# Autodesk Inventor assembly: Wheel
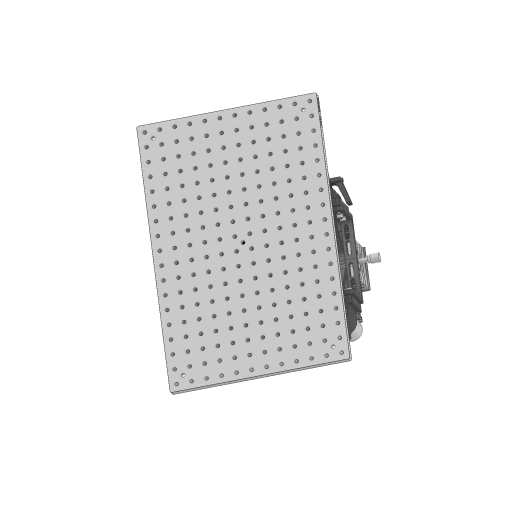
[picture p0: Inventor's stored thumbnail of the model, 512x512]
Saved by Autodesk Inventor 2024.1 (Build 281209000, 209)
## iProperties
Created: 2021-11-12
Part Number: Wheel
Document SubType Name: Assembly
Designer: gnzak
Author: gnzak
Comments: Wheel (spokes, track, clamp, axle, bearings): 0.306 lb Top Gonio: 0.661 Pillar: 3.73 Adjustable clamp: 1.09 3 5" t-slot rails: 0.624 brackets: 0.273 head bars: 1.02 wheel: 0.306 Total: 7.704 lb Max Capacity of bottom gonio: 6.61 16% over capacity
## Documents named in this file (29)
- C:\Users\rosam\Documents\repos\vr-frame-l7.033\Assemblies\Wheel_on-board_rotatable_original-headbars_adjustable.iam
- C:\Users\rosam\Documents\repos\vr-frame-l7.033\Parts\ThorLabs RA180\RA180.ipt
- C:\Users\rosam\Documents\repos\vr-frame-l7.033\Parts\ThorLabs PH1\PH1.ipt
- C:\Users\rosam\Documents\repos\vr-frame-l7.033\Parts\ThorLabs MB1218\MB1218 - Aluminium Breadboard 304.8 x 457.2 x 12.7mm_MB3030_M-1.ipt
- C:\Users\rosam\Documents\repos\vr-frame-l7.033\Parts\McMaster-Carr 47065T595\47065T595_Red Plastic Pull Handle.ipt
- C:\Users\rosam\Documents\repos\vr-frame-l7.033\Parts\ThorLabs TR6\TR6-Step.ipt
- C:\Users\rosam\Documents\repos\vr-frame-l7.033\Parts\ThorLabs TR12\TR12-Step.ipt
- C:\Users\rosam\Documents\repos\vr-frame-l7.033\Parts\ThorLabs TR2\TR2.ipt
- C:\Users\rosam\Documents\repos\vr-frame-l7.033\Parts\ThorLabs TR3\TR3-Step.ipt
- C:\Users\rosam\Documents\repos\vr-frame-l7.033\Parts\ThorLabs RA90\RA90-Step.ipt
- C:\Users\rosam\Documents\repos\vr-frame-l7.033\Parts\ThorLabs VH1\VH1-Step.ipt
- C:\Users\rosam\Documents\repos\vr-frame-l7.033\Parts\Parker Series 3 - Miniature Inert Liquid Valve\Series 3 (2way, .062Barb)-shell.ipt
- C:\Users\rosam\Documents\repos\vr-frame-l7.033\Parts\Solenoid Holder\Solenoid Mounting Panel.ipt
- C:\Users\rosam\Documents\repos\vr-frame-l7.033\Parts\McMaster-Carr 47065T801\47065T801_T-Slotted Framing_5-inches.ipt
- C:\Users\rosam\Documents\repos\vr-frame-l7.033\Parts\McMaster-Carr 47065T236\47065T236_Silver Corner Bracket.ipt
- C:\Users\rosam\Documents\repos\vr-frame-l7.033\Assemblies\Goniometers_70x70.iam
- C:\Users\rosam\Documents\repos\vr-frame-l7.033\Parts\Thorlabs C1515\C1515.ipt
- C:\Users\rosam\Documents\repos\vr-frame-l7.033\Parts\ThorLabs DP8A\DP8A-Step.ipt
- C:\Users\rosam\Documents\repos\vr-frame-l7.033\Parts\McMaster-Carr 47065T239\47065T239_Silver Corner Bracket.ipt
- C:\Users\rosam\Documents\repos\vr-frame-l7.033\Parts\McMaster-Carr 3136N157\3136N157_T-Slotted Framing.ipt
- C:\Users\rosam\Documents\repos\vr-frame-l7.033\Parts\McMaster-Carr 3136N175\3136N175_T-Slotted Framing.ipt
- C:\Users\rosam\Documents\repos\vr-frame-l7.033\Assemblies\Wheel.iam
- C:\Users\rosam\Documents\repos\vr-frame-l7.033\Parts\McMaster-Carr 47065T801\47065T801_T-Slotted Framing_4.4-inches.ipt
- C:\Users\rosam\Documents\repos\vr-frame-l7.033\Parts\McMaster-Carr 47065T255\47065T255_T-Slotted Framing.ipt
- C:\Users\rosam\Documents\repos\vr-frame-l7.033\Assemblies\bearing holder w bearing (vr).iam
- C:\Users\rosam\Documents\repos\vr-frame-l7.033\Assemblies\VR Head Bar Holder Left.iam
- C:\Users\rosam\Documents\repos\vr-frame-l7.033\Assemblies\VR Head Bar Holder Right.iam
- C:\Users\rosam\Documents\repos\vr-frame-l7.033\Parts\McMaster_Shaft-Coupler_6412K11\Shaft-Coupler_6412K11.ipt
- C:\Users\rosam\Documents\repos\vr-frame-l7.033\Parts\McMaster_Rotary-Shaft\6061K101_Linear Motion Shaft.ipt
## Components (44 placed, 28 different names)
1. MB1218 - Aluminium Breadboard 304.8 x 457.2 x 12.7mm_MB3030_M-1:1 — Angle:1, Mate:54, Mate:55, Mate:56, Mate:58, Mate:59, Mate:83, Mate:85, Mate:89, Angle:4, Angle:7, Mate:98, Angle:12, Angle:27, Mate:155, Mate:193, Mate:194, Angle:34, Angle:35, Mate:254, Mate:255, Mate:256, Angle:38, Angle:41, Mate:274, Mate:309, Angle:49, Mate:310, Angle:50
2. 47065T595_Red Plastic Pull Handle:1 — Mate:54, Mate:56, Mate:57, Mate:59
3. 47065T595_Red Plastic Pull Handle:2 — Mate:55, Mate:57, Mate:58
4. PH1:3 — Mate:85, Mate:89, Angle:7, Mate:97
5. PH1:5 — Mate:83, Angle:4, Mate:153, Mate:154
6. TR6-Step:4 — Mate:106, Mate:107, Mate:153, Mate:154, Mate:155
7. TR12-Step:1 — Mate:95, Mate:96, Mate:97, Mate:98
8. TR2:1 — Mate:95, Mate:96, Mate:99, Mate:100
9. RA180:3 — Mate:99, Mate:100, Mate:101, Mate:102, Angle:9, Angle:10
10. TR3-Step:1 — Mate:101, Mate:102, Mate:103, Flush:9, Mate:104, Flush:10
11. RA90-Step:1 — Mate:104, Flush:10, Angle:10
12. RA90-Step:2 — Mate:103, Flush:9, Angle:9, Angle:27
13. VH1-Step:1 — Mate:106, Angle:12, Mate:107
14. Series 3 (2way, .062Barb)-shell:3 — Mate:134, Angle:25, Mate:136, Mate:199
15. Series 3 (2way, .062Barb)-shell:4 — Mate:133, Mate:135, Angle:24, Mate:200
16. Solenoid Mounting Panel:2 — Mate:133, Mate:134, Mate:135, Angle:24, Angle:25, Mate:136, Mate:195, Mate:196, Angle:35
17. 47065T801_T-Slotted Framing_5-inches:1 — Mate:193, Mate:194, Angle:34, Mate:195, Mate:196, Mate:197, Mate:198, Flush:29, Flush:30
18. 47065T236_Silver Corner Bracket:1 — Mate:197, Mate:200, Flush:30
19. 47065T236_Silver Corner Bracket:2 — Mate:198, Mate:199, Flush:29
20. Goniometers_70x70:1 [sub-assembly] — Angle:38, Mate:262, Mate:276, Mate:277, Mate:280, Mate:281, Mate:282, Mate:303, Mate:305, Flush:78
21. 47065T801_T-Slotted Framing_5-inches:2 — Mate:248, Mate:252, Flush:47, Mate:298, Flush:57, Flush:58, Flush:62, Mate:302, Flush:63, Flush:64, Mate:316, Flush:71, Flush:72, Mate:321, Mate:325
22. 47065T801_T-Slotted Framing_5-inches:3 — Mate:250, Mate:253, Flush:49, Mate:299, Flush:59, Flush:60, Flush:61, Mate:314, Flush:67, Flush:68, Mate:315, Flush:69, Flush:70, Mate:323, Flush:79
23. C1515:2 — Mate:241, Flush:51, Mate:275, Flush:52, Mate:280, Flush:76
24. DP8A-Step:1 — Mate:241, Mate:254, Mate:255, Mate:256, Flush:76
25. 47065T239_Silver Corner Bracket:1 — Mate:248, Mate:298, Flush:57, Flush:58
26. 47065T239_Silver Corner Bracket:2 — Mate:250, Mate:299, Flush:59, Flush:60
27. 3136N157_T-Slotted Framing:1 — Mate:252, Flush:47, Flush:62, Mate:322
28. 3136N157_T-Slotted Framing:2 — Mate:253, Flush:49, Flush:61, Mate:324
29. 3136N175_T-Slotted Framing:1 — Mate:262, Mate:276, Mate:277, Mate:304
30. Wheel:1 [sub-assembly] — Tangent:1, Tangent:2, Flush:78
31. C1515:3 — Angle:41, Flush:51, Mate:275, Flush:52, Mate:281, Mate:282
32. DP8A-Step:2 — Mate:274
33. 47065T801_T-Slotted Framing_4.4-inches:1 — Mate:302, Flush:63, Flush:64, Mate:303, Mate:304, Mate:305, Mate:314, Flush:67, Flush:68
34. VH1-Step:2 — Mate:312, Mate:313
35. 47065T255_T-Slotted Framing:1 — Mate:309, Angle:49, Mate:310, Mate:311, Flush:65, Flush:66
36. 47065T801_T-Slotted Framing_5-inches:6 — Mate:311, Flush:65, Flush:66, Mate:312, Mate:313
37. 47065T801_T-Slotted Framing_5-inches:7 — Mate:316, Flush:71, Flush:72, Mate:317, Flush:73
38. 47065T801_T-Slotted Framing_5-inches:8 — Mate:315, Flush:69, Flush:70, Mate:318, Flush:74
39. bearing holder w bearing (vr):1 [sub-assembly] — Mate:317, Flush:73, Flush:75, Mate:327, Flush:80
40. bearing holder w bearing (vr):2 [sub-assembly] — Mate:318, Flush:74, Flush:75, Mate:326
41. VR Head Bar Holder Left:1 [sub-assembly] — Mate:321, Mate:322, Mate:325
42. VR Head Bar Holder Right:1 [sub-assembly] — Mate:323, Mate:324, Flush:79, Mate:326
43. Shaft-Coupler_6412K11:1 — Mate:328, Angle:50, Flush:81
44. 6061K101_Linear Motion Shaft:1 — Mate:327, Flush:80, Mate:328, Flush:81
## Relationships (131: Mate 79, Flush 33, Angle 17, Tangent 2)
- Angle:1 (0 deg): MB1218 - Aluminium Breadboard 304.8 x 457.2 x 12.7mm_MB3030_M-1:1
- Flush:6 (25.4 mm)
- Mate:54: MB1218 - Aluminium Breadboard 304.8 x 457.2 x 12.7mm_MB3030_M-1:1 ↔ 47065T595_Red Plastic Pull Handle:1
- Mate:55: MB1218 - Aluminium Breadboard 304.8 x 457.2 x 12.7mm_MB3030_M-1:1 ↔ 47065T595_Red Plastic Pull Handle:2
- Mate:56: MB1218 - Aluminium Breadboard 304.8 x 457.2 x 12.7mm_MB3030_M-1:1 ↔ 47065T595_Red Plastic Pull Handle:1
- Mate:57: 47065T595_Red Plastic Pull Handle:1 ↔ 47065T595_Red Plastic Pull Handle:2
- Mate:58 (-12.7 mm): MB1218 - Aluminium Breadboard 304.8 x 457.2 x 12.7mm_MB3030_M-1:1 ↔ 47065T595_Red Plastic Pull Handle:2
- Mate:59 (-12.7 mm): MB1218 - Aluminium Breadboard 304.8 x 457.2 x 12.7mm_MB3030_M-1:1 ↔ 47065T595_Red Plastic Pull Handle:1
- Mate:83: MB1218 - Aluminium Breadboard 304.8 x 457.2 x 12.7mm_MB3030_M-1:1 ↔ PH1:5
- Mate:85: MB1218 - Aluminium Breadboard 304.8 x 457.2 x 12.7mm_MB3030_M-1:1 ↔ PH1:3
- Mate:89: MB1218 - Aluminium Breadboard 304.8 x 457.2 x 12.7mm_MB3030_M-1:1 ↔ PH1:3
- Angle:4 (0 deg): MB1218 - Aluminium Breadboard 304.8 x 457.2 x 12.7mm_MB3030_M-1:1 ↔ PH1:5
- Angle:7 (0 deg): MB1218 - Aluminium Breadboard 304.8 x 457.2 x 12.7mm_MB3030_M-1:1 ↔ PH1:3
- Mate:95: TR12-Step:1 ↔ TR2:1
- Mate:96: TR12-Step:1 ↔ TR2:1
- Mate:97: PH1:3 ↔ TR12-Step:1
- Mate:98: MB1218 - Aluminium Breadboard 304.8 x 457.2 x 12.7mm_MB3030_M-1:1 ↔ TR12-Step:1
- Mate:99: TR2:1 ↔ RA180:3
- Mate:100: TR2:1 ↔ RA180:3
- Mate:101: RA180:3 ↔ TR3-Step:1
- Mate:102: RA180:3 ↔ TR3-Step:1
- Mate:103: TR3-Step:1 ↔ RA90-Step:2
- Flush:9: TR3-Step:1 ↔ RA90-Step:2
- Angle:9 (0 deg): RA180:3 ↔ RA90-Step:2
- Mate:104: TR3-Step:1 ↔ RA90-Step:1
- Flush:10: TR3-Step:1 ↔ RA90-Step:1
- Angle:10 (0 deg): RA180:3 ↔ RA90-Step:1
- Mate:106: TR6-Step:4 ↔ VH1-Step:1
- Angle:12 (0 deg): MB1218 - Aluminium Breadboard 304.8 x 457.2 x 12.7mm_MB3030_M-1:1 ↔ VH1-Step:1
- Mate:107: TR6-Step:4 ↔ VH1-Step:1
- [Mate]: Series 3 (2way, .062Barb)-shell:4 ↔ Solenoid Mounting Panel:2
- [Mate]: Series 3 (2way, .062Barb)-shell:3 ↔ Solenoid Mounting Panel:2
- [Angle] (0 deg): Series 3 (2way, .062Barb)-shell:4 ↔ Solenoid Mounting Panel:2
- [Angle] (0 deg): Series 3 (2way, .062Barb)-shell:3 ↔ Solenoid Mounting Panel:2
- Mate:133: Series 3 (2way, .062Barb)-shell:4 ↔ Solenoid Mounting Panel:2
- Mate:134: Series 3 (2way, .062Barb)-shell:3 ↔ Solenoid Mounting Panel:2
- Mate:135: Series 3 (2way, .062Barb)-shell:4 ↔ Solenoid Mounting Panel:2
- Angle:24 (0 deg): Series 3 (2way, .062Barb)-shell:4 ↔ Solenoid Mounting Panel:2
- Angle:25 (0 deg): Series 3 (2way, .062Barb)-shell:3 ↔ Solenoid Mounting Panel:2
- Mate:136: Series 3 (2way, .062Barb)-shell:3 ↔ Solenoid Mounting Panel:2
- Angle:27 (0 deg): MB1218 - Aluminium Breadboard 304.8 x 457.2 x 12.7mm_MB3030_M-1:1 ↔ RA90-Step:2
- Mate:153: PH1:5 ↔ TR6-Step:4
- Mate:154: PH1:5 ↔ TR6-Step:4
- Mate:155: MB1218 - Aluminium Breadboard 304.8 x 457.2 x 12.7mm_MB3030_M-1:1 ↔ TR6-Step:4
- Mate:193: MB1218 - Aluminium Breadboard 304.8 x 457.2 x 12.7mm_MB3030_M-1:1 ↔ 47065T801_T-Slotted Framing_5-inches:1
- Mate:194: MB1218 - Aluminium Breadboard 304.8 x 457.2 x 12.7mm_MB3030_M-1:1 ↔ 47065T801_T-Slotted Framing_5-inches:1
- Angle:34 (0 deg): MB1218 - Aluminium Breadboard 304.8 x 457.2 x 12.7mm_MB3030_M-1:1 ↔ 47065T801_T-Slotted Framing_5-inches:1
- Mate:195: Solenoid Mounting Panel:2 ↔ 47065T801_T-Slotted Framing_5-inches:1
- Mate:196: Solenoid Mounting Panel:2 ↔ 47065T801_T-Slotted Framing_5-inches:1
- Angle:35 (0 deg): MB1218 - Aluminium Breadboard 304.8 x 457.2 x 12.7mm_MB3030_M-1:1 ↔ Solenoid Mounting Panel:2
- Mate:197: 47065T801_T-Slotted Framing_5-inches:1 ↔ 47065T236_Silver Corner Bracket:1
- Mate:198: 47065T801_T-Slotted Framing_5-inches:1 ↔ 47065T236_Silver Corner Bracket:2
- Mate:199: Series 3 (2way, .062Barb)-shell:3 ↔ 47065T236_Silver Corner Bracket:2
- Flush:29: 47065T801_T-Slotted Framing_5-inches:1 ↔ 47065T236_Silver Corner Bracket:2
- Mate:200: Series 3 (2way, .062Barb)-shell:4 ↔ 47065T236_Silver Corner Bracket:1
- Flush:30: 47065T801_T-Slotted Framing_5-inches:1 ↔ 47065T236_Silver Corner Bracket:1
- Mate:241: C1515:2 ↔ DP8A-Step:1
- Mate:248: 47065T801_T-Slotted Framing_5-inches:2 ↔ 47065T239_Silver Corner Bracket:1
- Mate:250: 47065T801_T-Slotted Framing_5-inches:3 ↔ 47065T239_Silver Corner Bracket:2
- Mate:252: 47065T801_T-Slotted Framing_5-inches:2 ↔ 3136N157_T-Slotted Framing:1
- Flush:47: 47065T801_T-Slotted Framing_5-inches:2 ↔ 3136N157_T-Slotted Framing:1
- Mate:253: 47065T801_T-Slotted Framing_5-inches:3 ↔ 3136N157_T-Slotted Framing:2
- Flush:49: 47065T801_T-Slotted Framing_5-inches:3 ↔ 3136N157_T-Slotted Framing:2
- Mate:254: MB1218 - Aluminium Breadboard 304.8 x 457.2 x 12.7mm_MB3030_M-1:1 ↔ DP8A-Step:1
- Mate:255: MB1218 - Aluminium Breadboard 304.8 x 457.2 x 12.7mm_MB3030_M-1:1 ↔ DP8A-Step:1
- Mate:256: MB1218 - Aluminium Breadboard 304.8 x 457.2 x 12.7mm_MB3030_M-1:1 ↔ DP8A-Step:1
- Angle:38 (0 deg): MB1218 - Aluminium Breadboard 304.8 x 457.2 x 12.7mm_MB3030_M-1:1 ↔ Goniometers_70x70:1
- Mate:262: Goniometers_70x70:1 ↔ 3136N175_T-Slotted Framing:1
- Tangent:1: Wheel:1
- [Mate]: C1515:3 ↔ DP8A-Step:2
- Angle:41 (0 deg): MB1218 - Aluminium Breadboard 304.8 x 457.2 x 12.7mm_MB3030_M-1:1 ↔ C1515:3
- Mate:274: MB1218 - Aluminium Breadboard 304.8 x 457.2 x 12.7mm_MB3030_M-1:1 ↔ DP8A-Step:2
- Flush:51: C1515:2 ↔ C1515:3
- Mate:275: C1515:2 ↔ C1515:3
- Flush:52: C1515:2 ↔ C1515:3
- Mate:276: Goniometers_70x70:1 ↔ 3136N175_T-Slotted Framing:1
- Mate:277: Goniometers_70x70:1 ↔ 3136N175_T-Slotted Framing:1
- Tangent:2: Wheel:1
- Mate:280: Goniometers_70x70:1 ↔ C1515:2
- Mate:281: Goniometers_70x70:1 ↔ C1515:3
- Mate:282: Goniometers_70x70:1 ↔ C1515:3
- Mate:298: 47065T801_T-Slotted Framing_5-inches:2 ↔ 47065T239_Silver Corner Bracket:1
- Flush:57 (25.4 mm): 47065T801_T-Slotted Framing_5-inches:2 ↔ 47065T239_Silver Corner Bracket:1
- Flush:58 (2.54 mm): 47065T801_T-Slotted Framing_5-inches:2 ↔ 47065T239_Silver Corner Bracket:1
- Mate:299: 47065T801_T-Slotted Framing_5-inches:3 ↔ 47065T239_Silver Corner Bracket:2
- Flush:59 (25.4 mm): 47065T801_T-Slotted Framing_5-inches:3 ↔ 47065T239_Silver Corner Bracket:2
- Flush:60 (2.54 mm): 47065T801_T-Slotted Framing_5-inches:3 ↔ 47065T239_Silver Corner Bracket:2
- Flush:61: 47065T801_T-Slotted Framing_5-inches:3 ↔ 3136N157_T-Slotted Framing:2
- Flush:62: 47065T801_T-Slotted Framing_5-inches:2 ↔ 3136N157_T-Slotted Framing:1
- Mate:302: 47065T801_T-Slotted Framing_5-inches:2 ↔ 47065T801_T-Slotted Framing_4.4-inches:1
- Flush:63: 47065T801_T-Slotted Framing_5-inches:2 ↔ 47065T801_T-Slotted Framing_4.4-inches:1
- Flush:64: 47065T801_T-Slotted Framing_5-inches:2 ↔ 47065T801_T-Slotted Framing_4.4-inches:1
- Mate:303: Goniometers_70x70:1 ↔ 47065T801_T-Slotted Framing_4.4-inches:1
- Mate:304: 3136N175_T-Slotted Framing:1 ↔ 47065T801_T-Slotted Framing_4.4-inches:1
- Mate:305: Goniometers_70x70:1 ↔ 47065T801_T-Slotted Framing_4.4-inches:1
- Mate:309: MB1218 - Aluminium Breadboard 304.8 x 457.2 x 12.7mm_MB3030_M-1:1 ↔ 47065T255_T-Slotted Framing:1
- Angle:49 (0 deg): MB1218 - Aluminium Breadboard 304.8 x 457.2 x 12.7mm_MB3030_M-1:1 ↔ 47065T255_T-Slotted Framing:1
- Mate:310: MB1218 - Aluminium Breadboard 304.8 x 457.2 x 12.7mm_MB3030_M-1:1 ↔ 47065T255_T-Slotted Framing:1
- Mate:311: 47065T255_T-Slotted Framing:1 ↔ 47065T801_T-Slotted Framing_5-inches:6
- Flush:65: 47065T255_T-Slotted Framing:1 ↔ 47065T801_T-Slotted Framing_5-inches:6
- Flush:66: 47065T255_T-Slotted Framing:1 ↔ 47065T801_T-Slotted Framing_5-inches:6
- Mate:312: VH1-Step:2 ↔ 47065T801_T-Slotted Framing_5-inches:6
- Mate:313: VH1-Step:2 ↔ 47065T801_T-Slotted Framing_5-inches:6
- Mate:314: 47065T801_T-Slotted Framing_5-inches:3 ↔ 47065T801_T-Slotted Framing_4.4-inches:1
- Flush:67: 47065T801_T-Slotted Framing_5-inches:3 ↔ 47065T801_T-Slotted Framing_4.4-inches:1
- Flush:68: 47065T801_T-Slotted Framing_5-inches:3 ↔ 47065T801_T-Slotted Framing_4.4-inches:1
- Mate:315: 47065T801_T-Slotted Framing_5-inches:3 ↔ 47065T801_T-Slotted Framing_5-inches:8
- Flush:69: 47065T801_T-Slotted Framing_5-inches:3 ↔ 47065T801_T-Slotted Framing_5-inches:8
- Flush:70: 47065T801_T-Slotted Framing_5-inches:3 ↔ 47065T801_T-Slotted Framing_5-inches:8
- Mate:316: 47065T801_T-Slotted Framing_5-inches:2 ↔ 47065T801_T-Slotted Framing_5-inches:7
- Flush:71: 47065T801_T-Slotted Framing_5-inches:2 ↔ 47065T801_T-Slotted Framing_5-inches:7
- Flush:72: 47065T801_T-Slotted Framing_5-inches:2 ↔ 47065T801_T-Slotted Framing_5-inches:7
- Mate:317: 47065T801_T-Slotted Framing_5-inches:7 ↔ bearing holder w bearing (vr):1
- Flush:73 (6.35 mm): 47065T801_T-Slotted Framing_5-inches:7 ↔ bearing holder w bearing (vr):1
- Mate:318: 47065T801_T-Slotted Framing_5-inches:8 ↔ bearing holder w bearing (vr):2
- Flush:74 (6.35 mm): 47065T801_T-Slotted Framing_5-inches:8 ↔ bearing holder w bearing (vr):2
- Flush:75: bearing holder w bearing (vr):1 ↔ bearing holder w bearing (vr):2
- Flush:76 (50.8 mm): C1515:2 ↔ DP8A-Step:1
- Flush:78: Goniometers_70x70:1 ↔ Wheel:1
- Mate:321: 47065T801_T-Slotted Framing_5-inches:2 ↔ VR Head Bar Holder Left:1
- Mate:322: 3136N157_T-Slotted Framing:1 ↔ VR Head Bar Holder Left:1
- Mate:323: 47065T801_T-Slotted Framing_5-inches:3 ↔ VR Head Bar Holder Right:1
- Mate:324: 3136N157_T-Slotted Framing:2 ↔ VR Head Bar Holder Right:1
- Flush:79: 47065T801_T-Slotted Framing_5-inches:3 ↔ VR Head Bar Holder Right:1
- Mate:325: 47065T801_T-Slotted Framing_5-inches:2 ↔ VR Head Bar Holder Left:1
- Mate:326 (101.6 mm): bearing holder w bearing (vr):2 ↔ VR Head Bar Holder Right:1
- Mate:327: bearing holder w bearing (vr):1 ↔ 6061K101_Linear Motion Shaft:1
- Flush:80: bearing holder w bearing (vr):1 ↔ 6061K101_Linear Motion Shaft:1
- Mate:328: Shaft-Coupler_6412K11:1 ↔ 6061K101_Linear Motion Shaft:1
- Angle:50 (0 deg): MB1218 - Aluminium Breadboard 304.8 x 457.2 x 12.7mm_MB3030_M-1:1 ↔ Shaft-Coupler_6412K11:1
- Flush:81 (4.445 mm): Shaft-Coupler_6412K11:1 ↔ 6061K101_Linear Motion Shaft:1
## Named parameters: d226_d206 = 0 mm, d227_d207 = 0 mm, d229_d213 = 0 deg, d230_d214 = 0 deg, d512_d458 = 0 mm
